# Autodesk Inventor assembly: O ring dome Assembly
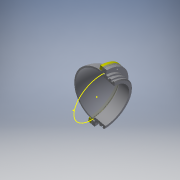
[picture p0: Inventor's stored thumbnail of the model, 180x180]
Saved by Autodesk Inventor 2016 (Build 200138000, 138)
## iProperties
Created: 2017-03-08
Part Number: O ring dome Assembly
Document SubType Name: Assembly
Designer: Student
Author: Student
## Documents named in this file (5)
- C:\Users\Student\Desktop\Noah Code\ROV\O ring dome Assembly.iam
- C:\Users\Student\Desktop\Noah Code\ROV\Oring Fitting Dome V2.ipt
- C:\Users\Student\Desktop\Noah Code\ROV\Oring Fitting Dome V2 -part.ipt
- C:\Users\Student\Desktop\Noah Code\ROV\4 inch PVC pipe.ipt
- C:\Users\Student\Desktop\Noah Code\ROV\ROV Dome 4'' (1).ipt
## Components (4 placed, 4 different names)
1. Oring Fitting Dome V2:1 — Rotational:1, Mate:1, Mate:3
2. Oring Fitting Dome V2 -part:1 — Mate:2, Mate:3
3. 4 inch PVC pipe:1
4. ROV Dome 4'' (1):1 — Rotational:1, Mate:1, Mate:2
## Relationships (4: Mate 3, RevoluteJoint 1)
- Rotational:1 [RevoluteJoint]: Oring Fitting Dome V2:1 ↔ ROV Dome 4'' (1):1
- Mate:1: Oring Fitting Dome V2:1 ↔ ROV Dome 4'' (1):1
- Mate:2: Oring Fitting Dome V2 -part:1 ↔ ROV Dome 4'' (1):1
- Mate:3: Oring Fitting Dome V2:1 ↔ Oring Fitting Dome V2 -part:1
